# Autodesk Inventor assembly: Jointed-arm robot
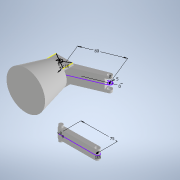
[picture p0: Inventor's stored thumbnail of the model, 180x180]
Saved by Autodesk Inventor 2020 (Build 240168000, 168)
## iProperties
Created: 2020-12-23
Part Number: Jointed-arm robot
Document SubType Name: Assembly
Designer: frost
Author: frost
## Documents named in this file (4)
- C:\Users\frost\OneDrive\Desktop\Intro to Robotics (1)\Jointed-arm robot.iam
- C:\Users\frost\OneDrive\Desktop\Intro to Robotics (1)\base.ipt
- C:\Users\frost\OneDrive\Desktop\Intro to Robotics (1)\shoulder swivel.ipt
- C:\Users\frost\OneDrive\Desktop\Intro to Robotics (1)\Elbow extension.ipt
## Components (3 placed, 3 different names)
1. base:1 — Insert:1
2. shoulder swivel:1 — Insert:1
3. Elbow extension:1
## Relationships (1: Insert 1)
- Insert:1: base:1 ↔ shoulder swivel:1
